# Autodesk Inventor assembly: prostkatna waska niska kwadraty
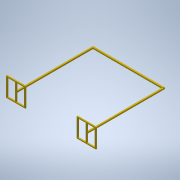
[picture p0: Inventor's stored thumbnail of the model, 180x180]
Saved by Autodesk Inventor 2021 (Build 250183000, 183)
## iProperties
Created: 2024-04-18
Part Number: prostkatna waska niska kwadraty
Document SubType Name: Assembly
Designer: Michal
Author: Michal
## Documents named in this file (6)
- C:\Users\Michal\Documents\GitHub\PNW_PhotoBoothFrame_3D\prostkatna waska niska kwadraty.iam
- C:\Users\Michal\Documents\GitHub\PNW_PhotoBoothFrame_3D\Gora L1500.ipt
- C:\Users\Michal\Documents\GitHub\PNW_PhotoBoothFrame_3D\Naroznik.iam
- C:\Users\Michal\Documents\GitHub\PNW_PhotoBoothFrame_3D\Stopa v1.iam
- C:\Users\Michal\Documents\GitHub\PNW_PhotoBoothFrame_3D\Noga L L1600.ipt
- C:\Users\Michal\Documents\GitHub\PNW_PhotoBoothFrame_3D\Noga P L1600.ipt
## Components (7 placed, 5 different names)
1. Stopa v1:1 [sub-assembly] — Flush:1, Flush:2, Mate:1, Flush:3, Mate:2
2. Stopa v1:2 [sub-assembly] — Flush:1, Flush:2, Mate:10, Flush:4, Flush:5, Mate:11
3. Naroznik:1 [sub-assembly] — Mate:12, Mate:13, Mate:14, Mate:15
4. Naroznik:2 [sub-assembly] — Mate:7, Mate:8, Mate:9, Mate:17
5. Noga L L1600:1 — Mate:1, Flush:3, Mate:2, Mate:7, Mate:8, Mate:9
6. Noga P L1600:1 — Mate:10, Flush:4, Flush:5, Mate:11, Mate:12, Mate:13, Mate:14, Flush:6
7. Gora L1500:1 — Flush:6, Mate:15, Mate:17, Mate:38, Flush:7, Mate:39
## Relationships (21: Mate 14, Flush 7)
- Flush:1: Stopa v1:1 ↔ Stopa v1:2
- Flush:2: Stopa v1:1 ↔ Stopa v1:2
- Mate:1: Stopa v1:1 ↔ Noga L L1600:1
- Flush:3: Stopa v1:1 ↔ Noga L L1600:1
- Mate:2: Stopa v1:1 ↔ Noga L L1600:1
- Mate:7: Naroznik:2 ↔ Noga L L1600:1
- Mate:8: Naroznik:2 ↔ Noga L L1600:1
- Mate:9: Naroznik:2 ↔ Noga L L1600:1
- Mate:10: Stopa v1:2 ↔ Noga P L1600:1
- Flush:4: Stopa v1:2 ↔ Noga P L1600:1
- Flush:5: Stopa v1:2 ↔ Noga P L1600:1
- Mate:11: Stopa v1:2 ↔ Noga P L1600:1
- Mate:12: Naroznik:1 ↔ Noga P L1600:1
- Mate:13: Naroznik:1 ↔ Noga P L1600:1
- Mate:14: Naroznik:1 ↔ Noga P L1600:1
- Flush:6: Noga P L1600:1 ↔ Gora L1500:1
- Mate:15: Naroznik:1 ↔ Gora L1500:1
- Mate:17: Naroznik:2 ↔ Gora L1500:1
- Mate:38: Gora L1500:1
- Flush:7: Gora L1500:1
- Mate:39: Gora L1500:1
